# Autodesk Inventor assembly: CraneAssembled
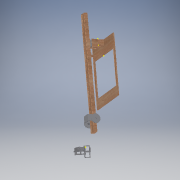
[picture p0: Inventor's stored thumbnail of the model, 180x180]
Saved by Autodesk Inventor 2016 (Build 200138000, 138)
## iProperties
Created: 2016-04-01
Part Number: CraneAssembled
Document SubType Name: Assembly
Designer: mkepler
Author: mkepler
## Documents named in this file (5)
- C:\Users\mkepler\Google Drive\Michael Kepler\College\ECE\ECE 590\Project 3\Physical Design\Inventor Files\CraneAssembled.iam
- C:\Users\mkepler\Google Drive\Michael Kepler\College\ECE\ECE 590\Project 3\Physical Design\Inventor Files\Trolley\Trolley.iam
- C:\Users\mkepler\Google Drive\Michael Kepler\College\ECE\ECE 590\Project 3\Physical Design\Inventor Files\Boom\BoomWithConnector.iam
- C:\Users\mkepler\Google Drive\Michael Kepler\College\ECE\ECE 590\Project 3\Physical Design\Inventor Files\Shaft\Shaft.iam
- C:\Users\mkepler\Google Drive\Michael Kepler\College\ECE\ECE 590\Project 3\Physical Design\Inventor Files\Claw\CLAW.iam
## Components (4 placed, 4 different names)
1. BoomWithConnector:1 [sub-assembly] — Insert:1, Insert:2, Mate:1, Mate:2, Mate:3, Insert:3
2. Shaft:1 [sub-assembly] — Insert:1, Insert:2, Insert:3
3. Trolley:1 [sub-assembly] — Mate:1, Mate:2, Mate:3
4. CLAW:1 [sub-assembly]
## Relationships (6: Insert 3, Mate 3)
- Insert:1: BoomWithConnector:1 ↔ Shaft:1
- Insert:2: BoomWithConnector:1 ↔ Shaft:1
- Mate:1: BoomWithConnector:1 ↔ Trolley:1
- Mate:2: BoomWithConnector:1 ↔ Trolley:1
- Mate:3: BoomWithConnector:1 ↔ Trolley:1
- Insert:3: BoomWithConnector:1 ↔ Shaft:1
